# Autodesk Inventor assembly: DYS SF2207 Brushless Motor v5 (2)
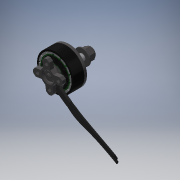
[picture p0: Inventor's stored thumbnail of the model, 180x180]
Saved by Autodesk Inventor 2019 (Build 230136000, 136)
## iProperties
Created: 2020-11-16
Part Number: DYS SF2207 Brushless Motor v5 (2)
Material: Ogólny
Document SubType Name: Assembly
Designer: Karol
Author: Karol
## Documents named in this file (4)
- C:\Users\Karol\Desktop\Koło naukowe KNMG\Drone\dys-sf2207-brushless-motor-1.snapshot.1\DYS SF2207 Brushless Motor v5 (2).iam
- C:\Users\Karol\Desktop\Koło naukowe KNMG\Drone\dys-sf2207-brushless-motor-1.snapshot.1\Base.ipt
- C:\Users\Karol\Desktop\Koło naukowe KNMG\Drone\dys-sf2207-brushless-motor-1.snapshot.1\Rotor.iam
- C:\Users\Karol\Desktop\Koło naukowe KNMG\Drone\dys-sf2207-brushless-motor-1.snapshot.1\Stator.iam
## Components (3 placed, 3 different names)
1. Base:1
2. Rotor:1 [sub-assembly]
3. Stator:1 [sub-assembly]
## Relationships (1: Flush 1)
- Równoległy:1 [Flush] (50 mm)
